# Autodesk Inventor assembly: Fingertip assembly final
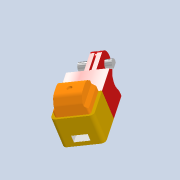
[picture p0: Inventor's stored thumbnail of the model, 180x180]
Saved by Autodesk Inventor 2020 (Build 240168000, 168)
## iProperties
Created: 2020-02-13
Part Number: Fingertip assembly final
Document SubType Name: Assembly
Designer: kaipa
Author: kaipa
## Documents named in this file (7)
- C:\Users\sami_\Documents\V1.6\Workgroups\NotInProject\MIDDLE\Fingertip assembly final.iam
- C:\Users\sami_\Documents\V1.6\Workgroups\NotInProject\MIDDLE\L3.ipt
- C:\Users\sami_\Documents\V1.6\Workgroups\NotInProject\MIDDLE\fingertip lid 5.ipt
- C:\Users\sami_\Documents\V1.6\Workgroups\NotInProject\MIDDLE\fingertip skeleton 5.ipt
- C:\Users\sami_\Documents\V1.6\Workgroups\NotInProject\MIDDLE\fingertip lid 5 no hole.ipt
- C:\Users\sami_\Documents\V1.6\Workgroups\NotInProject\SHAFT.ipt
- C:\Users\sami_\Documents\V1.6\Workgroups\NotInProject\Fingertiptest2-Solid 2mm base.ipt
## Components (6 placed, 6 different names)
1. fingertip lid 5:1 — Rigid:1
2. fingertip skeleton 5:1 — Rigid:1, Rigid:2, Rigid:3, Rigid:5
3. fingertip lid 5 no hole:1 — Rigid:2
4. L3:1 — Rigid:3
5. SHAFT:1
6. Fingertiptest2-Solid 2mm base:1 — Rigid:5
## Relationships (5: WeldJoint 5)
- Rigid:1 [WeldJoint]: fingertip lid 5:1 ↔ fingertip skeleton 5:1
- Rigid:2 [WeldJoint]: fingertip skeleton 5:1 ↔ fingertip lid 5 no hole:1
- Rigid:3 [WeldJoint]: fingertip skeleton 5:1 ↔ L3:1
- [WeldJoint] (3 mm): L3:1 ↔ SHAFT:1
- Rigid:5 [WeldJoint] (1 mm): fingertip skeleton 5:1 ↔ Fingertiptest2-Solid 2mm base:1
